# Autodesk Inventor assembly: Assembly1
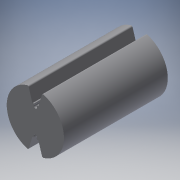
[picture p0: Inventor's stored thumbnail of the model, 180x180]
Saved by Autodesk Inventor 2017 (Build 210142000, 142)
## iProperties
Created: 2018-04-04
Part Number: Assembly1
Document SubType Name: Assembly
Designer: dasae
Author: dasae
## Documents named in this file (3)
- C:\Users\dasae\Documents\Work\Hiwi Neuroelectronic systems\CAD\heatsink\Assembly1.iam
- C:\Users\dasae\Documents\Work\Hiwi Neuroelectronic systems\CAD\heatsink\heatsink.ipt
- C:\Users\dasae\Documents\Work\Hiwi Neuroelectronic systems\CAD\heatsink\led.ipt
## Components (2 placed, 2 different names)
1. heatsink:1 — Mate:1, Mate:2
2. led:1 — Mate:1, Mate:2
## Relationships (2: Mate 2)
- Mate:1: heatsink:1 ↔ led:1
- Mate:2: heatsink:1 ↔ led:1
